# Autodesk Inventor assembly: chassis_2-02
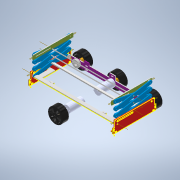
[picture p0: Inventor's stored thumbnail of the model, 180x180]
Saved by Autodesk Inventor 2022 (Build 260153000, 153)
## iProperties
Created: 2023-03-24
Part Number: chassis_2-02
Document SubType Name: Assembly
Designer: Johnny Jou
Author: Johnny Jou
## Documents named in this file (21)
- C:\Users\Johnny Jou\Documents\GitHub\Areo_Rider_Cabin\新增資料夾 (2)\新增資料夾 (2)\car\chassis_2.iam
- C:\Users\JOU\Desktop\git\Areo_Rider_Cabin\car\chassis_1_1.ipt
- C:\Users\Johnny Jou\Documents\GitHub\Areo_Rider_Cabin\新增資料夾 (2)\新增資料夾 (2)\car\chassis_1_2.ipt
- C:\Users\Johnny Jou\Documents\GitHub\Areo_Rider_Cabin\新增資料夾 (2)\新增資料夾 (2)\car\wheel.ipt
- C:\Users\Johnny Jou\Documents\GitHub\Areo_Rider_Cabin\新增資料夾 (2)\新增資料夾 (2)\car\wheel_base_cover.ipt
- C:\Users\Johnny Jou\Documents\GitHub\Areo_Rider_Cabin\新增資料夾 (2)\新增資料夾 (2)\car\bearing.iam
- C:\Users\Johnny Jou\Documents\GitHub\Areo_Rider_Cabin\新增資料夾 (2)\新增資料夾 (2)\car\axle 4_20.ipt
- C:\Users\Johnny Jou\Documents\GitHub\Areo_Rider_Cabin\新增資料夾 (2)\新增資料夾 (2)\car\Coupling.ipt
- C:\Users\Johnny Jou\Documents\GitHub\Areo_Rider_Cabin\新增資料夾 (2)\新增資料夾 (2)\Expansion\gasket.ipt
- C:\Users\Johnny Jou\Documents\GitHub\Areo_Rider_Cabin\新增資料夾 (2)\新增資料夾 (2)\Expansion\link_2022.ipt
- C:\Users\Johnny Jou\Documents\GitHub\Areo_Rider_Cabin\新增資料夾 (2)\新增資料夾 (2)\Expansion\rod_2.ipt
- C:\Users\Johnny Jou\Documents\GitHub\Areo_Rider_Cabin\新增資料夾 (2)\新增資料夾 (2)\car\chassis_1_1\chassis_1_1-02.ipt
- C:\Users\Johnny Jou\Documents\GitHub\Areo_Rider_Cabin\新增資料夾 (2)\新增資料夾 (2)\car\外抓檔\25GA370.ipt
- C:\Users\Johnny Jou\Documents\GitHub\Areo_Rider_Cabin\新增資料夾 (2)\新增資料夾 (2)\Expansion\rod_3.ipt
- C:\Users\Johnny Jou\Documents\GitHub\Areo_Rider_Cabin\新增資料夾 (2)\新增資料夾 (2)\car\chassis_1_4.ipt
- C:\Users\Johnny Jou\Documents\GitHub\Areo_Rider_Cabin\新增資料夾 (2)\新增資料夾 (2)\car\chassis_1_2_up.ipt
- C:\Users\Johnny Jou\Documents\GitHub\Areo_Rider_Cabin\car\chassis_2\AIP\FEA\eaz3jbjy8.fins
- C:\Users\Johnny Jou\Documents\GitHub\Areo_Rider_Cabin\car\chassis_2\AIP\FEA\eaz3jbjy8.fsat
- C:\Users\Johnny Jou\Documents\GitHub\Areo_Rider_Cabin\car\chassis_2\AIP\FEA\eaz3jbjy8.ftes
- C:\Users\Johnny Jou\Documents\GitHub\Areo_Rider_Cabin\car\chassis_2\AIP\FEA\eaz3jbjy8.fwiz
- C:\Users\Johnny Jou\Documents\GitHub\Areo_Rider_Cabin\car\chassis_2\AIP\FEA\eaz3jbk9s.fmsh
## Components (47 placed, 14 different names)
1. chassis_1_1-02:1 — 貼合:1, 齊平:1, 貼合:2, 齊平:2, 貼合:4, 貼合:5, 貼合:8, 貼合:9, 貼合:10, 貼合:14, 貼合:28, 貼合:29, 貼合:30, 貼合:31, 貼合:39, 貼合:40, 貼合:41
2. chassis_1_2:1 — 貼合:1, 齊平:1, 貼合:2, 貼合:62, 角度:1, 相切:2, 貼合:96, 貼合:97
3. chassis_1_2:2 — 齊平:2, 貼合:4, 貼合:5, 相切:1, 貼合:93, 貼合:95, 貼合:109
4. 25GA370:1 — 貼合:8, 貼合:9, 貼合:10, 貼合:11
5. Coupling:1 — 貼合:11, 貼合:12, 貼合:13, 貼合:14
6. wheel:1 — 貼合:12, 貼合:13
7. 25GA370:2
8. Coupling:2
9. wheel:2
10. Coupling:3 — 貼合:27, 貼合:28
11. wheel:3
12. 軸承:1 [sub-assembly] — 貼合:24, 貼合:25, 貼合:26, 齊平:4
13. wheel_base_cover:1 — 貼合:24, 貼合:25, 貼合:30, 貼合:31
14. axle 4_20:1 — 貼合:26, 齊平:4, 貼合:27, 貼合:29
15. Coupling:4 — 貼合:38
16. wheel:4
17. 軸承:2 [sub-assembly]
18. wheel_base_cover:2 — 貼合:38, 貼合:39, 貼合:40, 貼合:41
19. axle 4_20:2
20. 軸承:3 [sub-assembly]
21. 軸承:4 [sub-assembly]
22. rod_2:1 — 貼合:62, 角度:1, 貼合:63, 貼合:64, 貼合:65, 貼合:66, 貼合:94, 貼合:98
23. 軸承:5 [sub-assembly] — 貼合:63, 貼合:64, 相切:1
24. 軸承:6 [sub-assembly] — 貼合:65, 貼合:66, 相切:2
25. link_2022:1 — 貼合:67, up_and_down, 貼合:70, 貼合:71, 貼合:75, 貼合:94, 插入:3, 齊平:9, 貼合:100
26. link_2022:2 — 貼合:67, up_and_down, 貼合:70, 貼合:76, 貼合:91, 貼合:92, 貼合:93
27. link_2022:3 — 貼合:72, 貼合:76, 貼合:78, 齊平:8, 貼合:99
28. link_2022:4 — 貼合:71, 貼合:72, 貼合:73, 貼合:75, 貼合:77
29. link_2022:5 — 貼合:73, 貼合:74, 貼合:77, 齊平:10, 貼合:101, 插入:6
30. link_2022:6 — 貼合:74, 貼合:78, 貼合:112
31. link_2022:7 — 貼合:96, 貼合:97, 插入:2
32. link_2022:8 — 貼合:98, 插入:1
33. link_2022:9
34. link_2022:10
35. link_2022:11 — 貼合:113
36. link_2022:12 — 插入:4
37. gasket:1 — 貼合:91, 貼合:92, 貼合:95
38. gasket:2 — 插入:1
39. gasket:3 — 插入:2
40. gasket:4 — 插入:3
41. rod_3:1 — 齊平:8, 貼合:99
42. rod_3:2 — 齊平:9, 貼合:100
43. rod_3:3 — 齊平:10, 貼合:101
44. chassis_1_4:1 — 貼合:109
45. chassis_1_2_up:1 — 插入:5, 貼合:112
46. chassis_1_2_up:2 — 插入:4, 貼合:113
47. gasket:5 — 插入:5, 插入:6
## Relationships (99: Mate 77, Flush 7, Angle 7, Insert 6, Tangent 2)
- 貼合:1 [Mate]: chassis_1_1-02:1 ↔ chassis_1_2:1
- 齊平:1 [Flush]: chassis_1_1-02:1 ↔ chassis_1_2:1
- 貼合:2 [Mate]: chassis_1_1-02:1 ↔ chassis_1_2:1
- 齊平:2 [Flush]: chassis_1_1-02:1 ↔ chassis_1_2:2
- 貼合:4 [Mate]: chassis_1_1-02:1 ↔ chassis_1_2:2
- 貼合:5 [Mate]: chassis_1_1-02:1 ↔ chassis_1_2:2
- 貼合:8 [Mate]: chassis_1_1-02:1 ↔ 25GA370:1
- 貼合:9 [Mate]: chassis_1_1-02:1 ↔ 25GA370:1
- 貼合:10 [Mate]: chassis_1_1-02:1 ↔ 25GA370:1
- 貼合:11 [Mate]: 25GA370:1 ↔ Coupling:1
- 貼合:12 [Mate]: Coupling:1 ↔ wheel:1
- 貼合:13 [Mate]: Coupling:1 ↔ wheel:1
- 貼合:14 [Mate] (3 mm): chassis_1_1-02:1 ↔ Coupling:1
- [Mate]: 25GA370:2 ↔ Coupling:2
- [Mate]: Coupling:2 ↔ wheel:2
- [Mate]: Coupling:2 ↔ wheel:2
- [Mate]: Coupling:3 ↔ wheel:3
- [Mate]: Coupling:3 ↔ wheel:3
- 貼合:24 [Mate]: 軸承:1 ↔ wheel_base_cover:1
- 貼合:25 [Mate]: 軸承:1 ↔ wheel_base_cover:1
- 貼合:26 [Mate]: 軸承:1 ↔ axle 4_20:1
- 齊平:4 [Flush]: 軸承:1 ↔ axle 4_20:1
- 貼合:27 [Mate]: Coupling:3 ↔ axle 4_20:1
- 貼合:28 [Mate] (3 mm): chassis_1_1-02:1 ↔ Coupling:3
- 貼合:29 [Mate]: chassis_1_1-02:1 ↔ axle 4_20:1
- 貼合:30 [Mate]: chassis_1_1-02:1 ↔ wheel_base_cover:1
- 貼合:31 [Mate]: chassis_1_1-02:1 ↔ wheel_base_cover:1
- [Mate]: Coupling:4 ↔ wheel:4
- [Mate]: Coupling:4 ↔ wheel:4
- [Mate]: 軸承:2 ↔ wheel_base_cover:2
- [Mate]: 軸承:2 ↔ wheel_base_cover:2
- [Mate]: 軸承:2 ↔ axle 4_20:2
- [Flush]: 軸承:2 ↔ axle 4_20:2
- [Mate]: Coupling:4 ↔ axle 4_20:2
- 貼合:38 [Mate] (6 mm): Coupling:4 ↔ wheel_base_cover:2
- 貼合:39 [Mate]: chassis_1_1-02:1 ↔ wheel_base_cover:2
- 貼合:40 [Mate]: chassis_1_1-02:1 ↔ wheel_base_cover:2
- 貼合:41 [Mate]: chassis_1_1-02:1 ↔ wheel_base_cover:2
- 貼合:62 [Mate]: chassis_1_2:1 ↔ rod_2:1
- 角度:1 [Angle] (0 deg): chassis_1_2:1 ↔ rod_2:1
- 貼合:63 [Mate]: rod_2:1 ↔ 軸承:5
- 貼合:64 [Mate]: rod_2:1 ↔ 軸承:5
- 貼合:65 [Mate]: rod_2:1 ↔ 軸承:6
- 貼合:66 [Mate]: rod_2:1 ↔ 軸承:6
- 相切:1 [Tangent]: chassis_1_2:2 ↔ 軸承:5
- 相切:2 [Tangent]: chassis_1_2:1 ↔ 軸承:6
- 貼合:67 [Mate]: link_2022:1 ↔ link_2022:2
- up_and_down [Angle] (20 deg): link_2022:1 ↔ link_2022:2
- [Mate]: link_2022:3 ↔ link_2022:4
- [Angle] (20 deg): link_2022:3 ↔ link_2022:4
- [Mate]: link_2022:5 ↔ link_2022:6
- [Angle] (20 deg): link_2022:5 ↔ link_2022:6
- 貼合:70 [Mate]: link_2022:1 ↔ link_2022:2
- 貼合:71 [Mate]: link_2022:1 ↔ link_2022:4
- 貼合:72 [Mate]: link_2022:3 ↔ link_2022:4
- 貼合:73 [Mate]: link_2022:4 ↔ link_2022:5
- 貼合:74 [Mate]: link_2022:5 ↔ link_2022:6
- 貼合:75 [Mate]: link_2022:1 ↔ link_2022:4
- 貼合:76 [Mate]: link_2022:2 ↔ link_2022:3
- 貼合:77 [Mate]: link_2022:4 ↔ link_2022:5
- 貼合:78 [Mate]: link_2022:3 ↔ link_2022:6
- [Mate]: link_2022:7 ↔ link_2022:8
- [Angle] (20 deg): link_2022:7 ↔ link_2022:8
- [Mate]: link_2022:9 ↔ link_2022:10
- [Angle] (20 deg): link_2022:9 ↔ link_2022:10
- [Mate]: link_2022:11 ↔ link_2022:12
- [Angle] (20 deg): link_2022:11 ↔ link_2022:12
- [Mate]: link_2022:7 ↔ link_2022:8
- [Mate]: link_2022:7 ↔ link_2022:10
- [Mate]: link_2022:9 ↔ link_2022:10
- [Mate]: link_2022:10 ↔ link_2022:11
- [Mate]: link_2022:11 ↔ link_2022:12
- [Mate]: link_2022:7 ↔ link_2022:10
- [Mate]: link_2022:8 ↔ link_2022:9
- [Mate]: link_2022:10 ↔ link_2022:11
- [Mate]: link_2022:9 ↔ link_2022:12
- 貼合:91 [Mate]: link_2022:2 ↔ gasket:1
- 貼合:92 [Mate]: link_2022:2 ↔ gasket:1
- 貼合:93 [Mate]: chassis_1_2:2 ↔ link_2022:2
- 貼合:94 [Mate]: rod_2:1 ↔ link_2022:1
- 貼合:95 [Mate]: chassis_1_2:2 ↔ gasket:1
- 貼合:96 [Mate]: chassis_1_2:1 ↔ link_2022:7
- 貼合:97 [Mate]: chassis_1_2:1 ↔ link_2022:7
- 貼合:98 [Mate]: rod_2:1 ↔ link_2022:8
- 插入:1 [Insert]: link_2022:8 ↔ gasket:2
- 插入:2 [Insert]: link_2022:7 ↔ gasket:3
- 插入:3 [Insert]: link_2022:1 ↔ gasket:4
- 齊平:8 [Flush]: link_2022:3 ↔ rod_3:1
- 貼合:99 [Mate]: link_2022:3 ↔ rod_3:1
- 齊平:9 [Flush]: link_2022:1 ↔ rod_3:2
- 貼合:100 [Mate]: link_2022:1 ↔ rod_3:2
- 齊平:10 [Flush]: link_2022:5 ↔ rod_3:3
- 貼合:101 [Mate]: link_2022:5 ↔ rod_3:3
- 貼合:109 [Mate]: chassis_1_2:2 ↔ chassis_1_4:1
- 插入:4 [Insert]: link_2022:12 ↔ chassis_1_2_up:2
- 插入:5 [Insert]: chassis_1_2_up:1 ↔ gasket:5
- 插入:6 [Insert]: link_2022:5 ↔ gasket:5
- 貼合:112 [Mate]: link_2022:6 ↔ chassis_1_2_up:1
- 貼合:113 [Mate]: link_2022:11 ↔ chassis_1_2_up:2
## Named parameters: sa_0 = 137.2, d355_d351 = 0 mm, d356_d352 = 0 mm, d357_d353 = 0 mm, d362_d352 = 0 mm, d363_d353 = 0 mm, d373_d362_d352 = 0 mm, d374_d363_d353 = 0 mm, d375_d364 = 0 mm, d376_d365 = 0 mm, d377_d366 = 0 mm, d378_d367 = 0 mm, d379_d368 = 0 mm, d416_d414 = 0 mm, d417_d415 = 20 deg, d418_d414 = 0 mm, d419_d415 = 20 deg, d435_d424 = 0 mm, d436_d425 = 0 mm, d437_d426 = 0 mm, d438_d427 = 0 mm, d439_d428 = 0 mm, d440_d414 = 0 mm, d441_d415 = 20 deg, d442_d416_d414 = 0 mm, d444_d418_d414 = 0 mm, d446_d420 = 0 mm, d447_d421 = 0 mm, d448_d422 = 0 mm, d449_d423 = 0 mm
note: some values were not read from the file. Shown as the stored number, unit unknown: "sa_0".
